# Autodesk Inventor assembly: Assembly_WG_writer
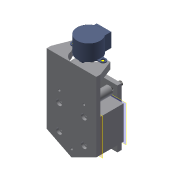
[picture p0: Inventor's stored thumbnail of the model, 180x180]
Saved by Autodesk Inventor 2019.4 (Build 234330000, 330)
## iProperties
Created: 2020-11-13
Part Number: Assembly_WG_writer
Document SubType Name: Assembly
Designer: diederichbenedict
Author: diederichbenedict
## Documents named in this file (7)
- C:\Users\diederichbenedict\Dropbox\Dokumente\Promotion\PROJECTS\STORMoChip\GITHUB\CAD\cellSTORM_inverted\Workspace\Assembly_WG_writer.iam
- C:\Users\diederichbenedict\Dropbox\Dokumente\Promotion\PROJECTS\STORMoChip\GITHUB\CAD\cellSTORM_inverted\Workspace\00_Z-stage.ipt
- C:\Users\diederichbenedict\Dropbox\Dokumente\Promotion\PROJECTS\STORMoChip\GITHUB\CAD\cellSTORM_inverted\Workspace\00_Stepper_Motor_28BYJ-48.0013.ipt
- C:\Users\diederichbenedict\Dropbox\Dokumente\Promotion\PROJECTS\STORMoChip\GITHUB\CAD\cellSTORM_inverted\Workspace\01_WG_writer_BASE.ipt
- C:\Users\diederichbenedict\Dropbox\Dokumente\Promotion\PROJECTS\STORMoChip\GITHUB\CAD\cellSTORM_inverted\Workspace\02_WG_writer_clutch.ipt
- C:\Users\diederichbenedict\Dropbox\Dokumente\Promotion\PROJECTS\STORMoChip\GITHUB\CAD\cellSTORM_inverted\Workspace\DIN 912 - M3 x 0.5 x 12 x 10.75.ipt
- C:\Users\diederichbenedict\Dropbox\Dokumente\Promotion\PROJECTS\STORMoChip\GITHUB\CAD\cellSTORM_inverted\Workspace\03_MountCoverslip.ipt
## Components (8 placed, 6 different names)
1. 00_Z-stage:1 — Insert:1, Flush:1, Flush:2, Flush:3, Flush:4, Flush:5
2. 00_Stepper_Motor_28BYJ-48.0013:1 — Insert:1
3. 01_WG_writer_BASE:1 — Flush:1, Flush:2, Insert:2, Insert:3, Insert:4
4. 02_WG_writer_clutch:1 — Flush:3
5. DIN 912 - replaced by DIN EN ISO 4762 M3 x 12:1 — Insert:2
6. DIN 912 - replaced by DIN EN ISO 4762 M3 x 12:2 — Insert:3
7. DIN 912 - replaced by DIN EN ISO 4762 M3 x 12:3 — Insert:4
8. 03_MountCoverslip:1 — Flush:4, Flush:5
## Relationships (9: Flush 5, Insert 4)
- Insert:1 (1 mm): 00_Z-stage:1 ↔ 00_Stepper_Motor_28BYJ-48.0013:1
- Flush:1: 00_Z-stage:1 ↔ 01_WG_writer_BASE:1
- Flush:2: 00_Z-stage:1 ↔ 01_WG_writer_BASE:1
- Flush:3: 00_Z-stage:1 ↔ 02_WG_writer_clutch:1
- Insert:2: 01_WG_writer_BASE:1 ↔ DIN 912 - replaced by DIN EN ISO 4762 M3 x 12:1
- Insert:3: 01_WG_writer_BASE:1 ↔ DIN 912 - replaced by DIN EN ISO 4762 M3 x 12:2
- Insert:4: 01_WG_writer_BASE:1 ↔ DIN 912 - replaced by DIN EN ISO 4762 M3 x 12:3
- Flush:4: 00_Z-stage:1 ↔ 03_MountCoverslip:1
- Flush:5: 00_Z-stage:1 ↔ 03_MountCoverslip:1
